# Autodesk Inventor assembly: Arm Assembly, Left
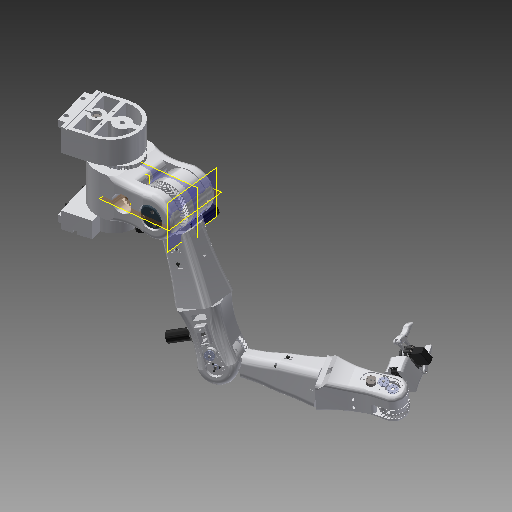
[picture p0: Inventor's stored thumbnail of the model, 512x512]
Saved by Autodesk Inventor 2017 (Build 210142000, 142)
## iProperties
Created: 2017-09-28
Part Number: Arm Assembly, Left
Document SubType Name: Assembly
Designer: Zach
Author: Zach
## Documents named in this file (7)
- C:\Users\Dell\Documents\GitHub\tr1\src\Body\Arm Assembly\Arm Assembly, Left.iam
- C:\Users\Dell\Documents\GitHub\tr1\src\Body\Arm Assembly\Bicep Assembly\Bicep Assembly.iam
- C:\Users\Dell\Documents\GitHub\tr1\src\Body\Arm Assembly\Forearm Assembly\Forearm Assembly.iam
- C:\Users\Dell\Documents\GitHub\tr1\src\Body\Arm Assembly\Elbow Assembly\Elbow Assembly.iam
- C:\Users\Dell\Documents\GitHub\tr1\src\Body\Arm Assembly\Wrist Assembly\Wrist Assembly.iam
- C:\Users\Dell\Documents\GitHub\tr1\src\Body\Arm Assembly\End Effector Assembly\End Effector Assembly.iam
- C:\Users\Dell\Documents\GitHub\tr1\src\Body\Arm Assembly\Shoulder Assembly\Shoulder Assembly, Left.iam
## Components (6 placed, 6 different names)
1. Shoulder Assembly, Left:1 [sub-assembly] — Mate:8, Flush:4
2. Bicep Assembly:1 [sub-assembly] — Mate:2, Mate:3, Mate:8, Flush:4
3. Forearm Assembly:1 [sub-assembly] — Mate:4, Flush:2, Mate:5, Mate:6
4. Elbow Assembly:1 [sub-assembly] — Mate:2, Mate:3, Mate:4, Flush:2
5. Wrist Assembly:1 [sub-assembly] — Mate:5, Mate:6, Mate:7, Flush:3
6. End Effector Assembly:1 [sub-assembly] — Mate:7, Flush:3
## Relationships (10: Mate 7, Flush 3)
- Mate:2: Bicep Assembly:1 ↔ Elbow Assembly:1
- Mate:3: Bicep Assembly:1 ↔ Elbow Assembly:1
- Mate:4: Forearm Assembly:1 ↔ Elbow Assembly:1
- Flush:2: Forearm Assembly:1 ↔ Elbow Assembly:1
- Mate:5: Forearm Assembly:1 ↔ Wrist Assembly:1
- Mate:6: Forearm Assembly:1 ↔ Wrist Assembly:1
- Mate:7: Wrist Assembly:1 ↔ End Effector Assembly:1
- Flush:3: Wrist Assembly:1 ↔ End Effector Assembly:1
- Mate:8: Shoulder Assembly, Left:1 ↔ Bicep Assembly:1
- Flush:4: Shoulder Assembly, Left:1 ↔ Bicep Assembly:1
